# Autodesk Inventor assembly: ZAxisRodsandGripper
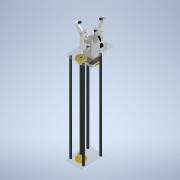
[picture p0: Inventor's stored thumbnail of the model, 180x180]
Saved by Autodesk Inventor 2022 (Build 260153000, 153)
## iProperties
Created: 2021-06-28
Part Number: ZAxisRodsandGripper
Document SubType Name: Assembly
Designer: domin
Author: domin
## Documents named in this file (17)
- E:\Transfer\Sync\Hivemind\1-MCI-Unterlagen\Master\Semester 3\Projekt 2\011_Kartesischer_Roboter_Modul\07-CAD Files\02-Kartesischer Roboter\ZAxisandGripper\ZAxisRodsandGripper.iam
- E:\Transfer\Sync\Hivemind\1-MCI-Unterlagen\Master\Semester 3\Projekt 2\011_Kartesischer_Roboter_Modul\07-CAD Files\02-Kartesischer Roboter\Einzelteile\Gripper_Base.ipt
- E:\Transfer\Sync\Hivemind\1-MCI-Unterlagen\Master\Semester 3\Projekt 2\011_Kartesischer_Roboter_Modul\07-CAD Files\02-Kartesischer Roboter\Einzelteile\Gripper_Outer_Support_2.ipt
- E:\Transfer\Sync\Hivemind\1-MCI-Unterlagen\Master\Semester 3\Projekt 2\011_Kartesischer_Roboter_Modul\07-CAD Files\02-Kartesischer Roboter\Einzelteile\Gripper_Outer_Support.ipt
- E:\Transfer\Sync\Hivemind\1-MCI-Unterlagen\Master\Semester 3\Projekt 2\011_Kartesischer_Roboter_Modul\07-CAD Files\02-Kartesischer Roboter\Einzelteile\Ender_Motor.ipt
- E:\Transfer\Sync\Hivemind\1-MCI-Unterlagen\Master\Semester 3\Projekt 2\011_Kartesischer_Roboter_Modul\07-CAD Files\02-Kartesischer Roboter\Einzelteile\Trapezmutter_T8_ganz.ipt
- E:\Transfer\Sync\Hivemind\1-MCI-Unterlagen\Master\Semester 3\Projekt 2\011_Kartesischer_Roboter_Modul\07-CAD Files\02-Kartesischer Roboter\Einzelteile\White_Cable_Tie_Mount_RS666-717.ipt
- E:\Transfer\Sync\Hivemind\1-MCI-Unterlagen\Master\Semester 3\Projekt 2\011_Kartesischer_Roboter_Modul\07-CAD Files\02-Kartesischer Roboter\Einzelteile\Bolt_3_23.ipt
- E:\Transfer\Sync\Hivemind\1-MCI-Unterlagen\Master\Semester 3\Projekt 2\011_Kartesischer_Roboter_Modul\07-CAD Files\02-Kartesischer Roboter\Einzelteile\Gripper_Spindle.iam
- E:\Transfer\Sync\Hivemind\1-MCI-Unterlagen\Master\Semester 3\Projekt 2\011_Kartesischer_Roboter_Modul\07-CAD Files\02-Kartesischer Roboter\Einzelteile\Gripper_Endstop_Holder.ipt
- E:\Transfer\Sync\Hivemind\1-MCI-Unterlagen\Master\Semester 3\Projekt 2\011_Kartesischer_Roboter_Modul\07-CAD Files\02-Kartesischer Roboter\Einzelteile\Endstop.ipt
- E:\Transfer\Sync\Hivemind\1-MCI-Unterlagen\Master\Semester 3\Projekt 2\011_Kartesischer_Roboter_Modul\07-CAD Files\02-Kartesischer Roboter\Einzelteile\Gripper_Central_Plate.ipt
- E:\Transfer\Sync\Hivemind\1-MCI-Unterlagen\Master\Semester 3\Projekt 2\011_Kartesischer_Roboter_Modul\07-CAD Files\02-Kartesischer Roboter\Einzelteile\Gripper_Arm.iam
- E:\Transfer\Sync\Hivemind\1-MCI-Unterlagen\Master\Semester 3\Projekt 2\011_Kartesischer_Roboter_Modul\07-CAD Files\02-Kartesischer Roboter\Einzelteile\Gripper_Link.iam
- E:\Transfer\Sync\Hivemind\1-MCI-Unterlagen\Master\Semester 3\Projekt 2\011_Kartesischer_Roboter_Modul\07-CAD Files\02-Kartesischer Roboter\Einzelteile\Z-Kettenhalter3.ipt
- E:\Transfer\Sync\Hivemind\1-MCI-Unterlagen\Master\Semester 3\Projekt 2\011_Kartesischer_Roboter_Modul\07-CAD Files\02-Kartesischer Roboter\Einzelteile\Stange_8mm_400mm.ipt
- E:\Transfer\Sync\Hivemind\1-MCI-Unterlagen\Master\Semester 3\Projekt 2\011_Kartesischer_Roboter_Modul\07-CAD Files\02-Kartesischer Roboter\Einzelteile\Z_platte_oben_new_8mm.ipt
## Components (30 placed, 16 different names)
1. Gripper_Base:1 — Flush:2, Mate:1, Flush:3, Mate:2, Mate:3, Mate:4, Mate:5, Mate:6, Mate:7, Mate:8, Mate:9, Mate:10, Mate:11, Mate:12, Angle:1, Mate:13, Mate:14, Mate:15, Mate:16, Mate:17, Angle:2, Mate:43, Mate:44, Mate:45, Mate:46, Mate:47, Mate:49, Mate:50, Mate:51, Mate:52, Mate:53, Angle:3, Flush:6, Flush:7
2. Gripper_Outer_Support_2:1 — Mate:2, Mate:3, Mate:4, Mate:18, Mate:21, Mate:35
3. Gripper_Outer_Support:1 — Mate:5, Mate:6, Mate:7, Mate:19, Flush:5, Mate:36, Mate:24, Mate:25, Mate:26
4. Gripper_Outer_Support:2 — Mate:8, Mate:9, Mate:10, Mate:20, Flush:4, Mate:37, Mate:27, Mate:28, Mate:60
5. Ender_Motor:1 — Mate:11, Mate:12, Angle:1, Mate:22, Mate:23
6. Trapezmutter_T8_ganz:1 — Mate:13, Mate:14, Mate:15, Mate:48
7. White_Cable_Tie_Mount_RS666-717:1 — Mate:16, Mate:17, Angle:2
8. Bolt_3_23:1 — Mate:18, Mate:21, Cylindrical:2
9. Bolt_3_23:2 — Mate:19, Flush:5, Cylindrical:3
10. Bolt_3_23:3 — Mate:20, Flush:4, Cylindrical:4
11. Gripper_Spindle:1 [sub-assembly] — Mate:22, Mate:23, Cylindrical:1
12. Gripper_Endstop_Holder:1 — Mate:24, Mate:25, Mate:26, Mate:29, Mate:30, Mate:31
13. Gripper_Endstop_Holder:2 — Mate:27, Mate:28, Mate:32, Mate:33, Mate:34, Mate:60
14. Endstop:1 — Mate:29, Mate:30, Mate:31
15. Endstop:2 — Mate:32, Mate:33, Mate:34
16. Gripper_Central_Plate:1 — Cylindrical:1, Cylindrical:8, Cylindrical:10, Cylindrical:12
17. Gripper_Arm:1 [sub-assembly] — Mate:35, Cylindrical:2, Mate:38, Cylindrical:5
18. Gripper_Arm:2 [sub-assembly] — Mate:36, Cylindrical:3, Mate:59, Cylindrical:9
19. Gripper_Arm:3 [sub-assembly] — Mate:37, Cylindrical:4, Mate:40, Cylindrical:11
20. Gripper_Link:1 [sub-assembly] — Mate:38, Cylindrical:5, Cylindrical:8
21. Gripper_Link:2 [sub-assembly] — Mate:59, Cylindrical:9, Cylindrical:10
22. Gripper_Link:3 [sub-assembly] — Mate:40, Cylindrical:11, Cylindrical:12
23. Z-Kettenhalter3:1 — Mate:43, Flush:6, Flush:7
24. Stange_8mm_400mm:1 — Mate:44, Mate:49
25. Stange_8mm_400mm:2 — Mate:45, Mate:50
26. Stange_8mm_400mm:3 — Mate:46, Mate:51
27. Stange_8mm_400mm:4 — Mate:47, Mate:52
28. Stange_8mm_400mm:5 — Mate:48, Mate:53, Mate:57, Mate:58
29. Z_platte_oben_new_8mm:1 — Mate:54, Mate:55, Mate:56, Mate:58, Angle:3
30. Trapezmutter_T8_ganz:2 — Mate:54, Mate:55, Mate:56, Mate:57
## Relationships (76: Mate 57, CylindricalJoint 10, Flush 6, Angle 3)
- Flush:2: Gripper_Base:1
- Mate:1: Gripper_Base:1
- Flush:3: Gripper_Base:1
- Mate:2: Gripper_Base:1 ↔ Gripper_Outer_Support_2:1
- Mate:3: Gripper_Base:1 ↔ Gripper_Outer_Support_2:1
- Mate:4: Gripper_Base:1 ↔ Gripper_Outer_Support_2:1
- Mate:5: Gripper_Base:1 ↔ Gripper_Outer_Support:1
- Mate:6: Gripper_Base:1 ↔ Gripper_Outer_Support:1
- Mate:7: Gripper_Base:1 ↔ Gripper_Outer_Support:1
- Mate:8: Gripper_Base:1 ↔ Gripper_Outer_Support:2
- Mate:9: Gripper_Base:1 ↔ Gripper_Outer_Support:2
- Mate:10: Gripper_Base:1 ↔ Gripper_Outer_Support:2
- Mate:11: Gripper_Base:1 ↔ Ender_Motor:1
- Mate:12: Gripper_Base:1 ↔ Ender_Motor:1
- Angle:1 (0 deg): Gripper_Base:1 ↔ Ender_Motor:1
- Mate:13: Gripper_Base:1 ↔ Trapezmutter_T8_ganz:1
- Mate:14: Gripper_Base:1 ↔ Trapezmutter_T8_ganz:1
- Mate:15: Gripper_Base:1 ↔ Trapezmutter_T8_ganz:1
- Mate:16: Gripper_Base:1 ↔ White_Cable_Tie_Mount_RS666-717:1
- Mate:17: Gripper_Base:1 ↔ White_Cable_Tie_Mount_RS666-717:1
- Angle:2 (0 deg): Gripper_Base:1 ↔ White_Cable_Tie_Mount_RS666-717:1
- Mate:18: Gripper_Outer_Support_2:1 ↔ Bolt_3_23:1
- Mate:19: Gripper_Outer_Support:1 ↔ Bolt_3_23:2
- Mate:20: Gripper_Outer_Support:2 ↔ Bolt_3_23:3
- Mate:21: Gripper_Outer_Support_2:1 ↔ Bolt_3_23:1
- Flush:4: Gripper_Outer_Support:2 ↔ Bolt_3_23:3
- Flush:5: Gripper_Outer_Support:1 ↔ Bolt_3_23:2
- Mate:22: Ender_Motor:1 ↔ Gripper_Spindle:1
- Mate:23 (3 mm): Ender_Motor:1 ↔ Gripper_Spindle:1
- Mate:24: Gripper_Outer_Support:1 ↔ Gripper_Endstop_Holder:1
- Mate:25: Gripper_Outer_Support:1 ↔ Gripper_Endstop_Holder:1
- Mate:26: Gripper_Outer_Support:1 ↔ Gripper_Endstop_Holder:1
- Mate:27: Gripper_Outer_Support:2 ↔ Gripper_Endstop_Holder:2
- Mate:28: Gripper_Outer_Support:2 ↔ Gripper_Endstop_Holder:2
- Mate:29: Gripper_Endstop_Holder:1 ↔ Endstop:1
- Mate:30: Gripper_Endstop_Holder:1 ↔ Endstop:1
- Mate:31: Gripper_Endstop_Holder:1 ↔ Endstop:1
- Mate:32: Gripper_Endstop_Holder:2 ↔ Endstop:2
- Mate:33: Gripper_Endstop_Holder:2 ↔ Endstop:2
- Mate:34: Gripper_Endstop_Holder:2 ↔ Endstop:2
- Cylindrical:1: Gripper_Spindle:1 ↔ Gripper_Central_Plate:1
- Mate:35: Gripper_Outer_Support_2:1 ↔ Gripper_Arm:1
- Mate:36: Gripper_Outer_Support:1 ↔ Gripper_Arm:2
- Mate:37: Gripper_Outer_Support:2 ↔ Gripper_Arm:3
- Cylindrical:2: Bolt_3_23:1 ↔ Gripper_Arm:1
- Cylindrical:3: Bolt_3_23:2 ↔ Gripper_Arm:2
- Cylindrical:4: Bolt_3_23:3 ↔ Gripper_Arm:3
- Mate:38 (0.5 mm): Gripper_Arm:1 ↔ Gripper_Link:1
- Mate:59 (0.5 mm): Gripper_Arm:2 ↔ Gripper_Link:2
- Mate:40 (0.5 mm): Gripper_Arm:3 ↔ Gripper_Link:3
- Cylindrical:5: Gripper_Arm:1 ↔ Gripper_Link:1
- Cylindrical:8: Gripper_Central_Plate:1 ↔ Gripper_Link:1
- Mate:43: Gripper_Base:1 ↔ Z-Kettenhalter3:1
- Mate:44: Gripper_Base:1 ↔ Stange_8mm_400mm:1
- Mate:45: Gripper_Base:1 ↔ Stange_8mm_400mm:2
- Mate:46: Gripper_Base:1 ↔ Stange_8mm_400mm:3
- Mate:47: Gripper_Base:1 ↔ Stange_8mm_400mm:4
- Mate:48: Trapezmutter_T8_ganz:1 ↔ Stange_8mm_400mm:5
- Mate:49: Gripper_Base:1 ↔ Stange_8mm_400mm:1
- Mate:50: Gripper_Base:1 ↔ Stange_8mm_400mm:2
- Mate:51: Gripper_Base:1 ↔ Stange_8mm_400mm:3
- Mate:52: Gripper_Base:1 ↔ Stange_8mm_400mm:4
- Mate:53: Gripper_Base:1 ↔ Stange_8mm_400mm:5
- Mate:54: Z_platte_oben_new_8mm:1 ↔ Trapezmutter_T8_ganz:2
- Mate:55: Z_platte_oben_new_8mm:1 ↔ Trapezmutter_T8_ganz:2
- Mate:56: Z_platte_oben_new_8mm:1 ↔ Trapezmutter_T8_ganz:2
- Mate:57: Stange_8mm_400mm:5 ↔ Trapezmutter_T8_ganz:2
- Mate:58: Stange_8mm_400mm:5 ↔ Z_platte_oben_new_8mm:1
- Angle:3 (0 deg): Gripper_Base:1 ↔ Z_platte_oben_new_8mm:1
- Cylindrical:9: Gripper_Arm:2 ↔ Gripper_Link:2
- Cylindrical:10: Gripper_Central_Plate:1 ↔ Gripper_Link:2
- Cylindrical:11: Gripper_Arm:3 ↔ Gripper_Link:3
- Cylindrical:12: Gripper_Central_Plate:1 ↔ Gripper_Link:3
- Mate:60: Gripper_Outer_Support:2 ↔ Gripper_Endstop_Holder:2
- Flush:6: Gripper_Base:1 ↔ Z-Kettenhalter3:1
- Flush:7 (-25 mm): Gripper_Base:1 ↔ Z-Kettenhalter3:1
